# Autodesk Inventor assembly: lançador
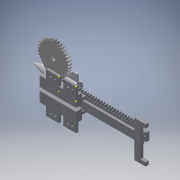
[picture p0: Inventor's stored thumbnail of the model, 180x180]
Saved by Autodesk Inventor 2019 (Build 230136000, 136)
## iProperties
Created: 2018-06-06
Part Number: lançador
Material: Genérico
Document SubType Name: Assembly
Designer: Ernandes
Author: Ernandes
## Documents named in this file (5)
- C:\Users\Ernandes\Google Drive (sguimaraaes@gmail.com)\TCC\3D\lançador.inventor\lançador.inventor\lançador.iam
- C:\Users\Ernandes\Google Drive (sguimaraaes@gmail.com)\TCC\3D\lançador.inventor\lançador.inventor\cremalheira pronta.iam
- C:\Users\Ernandes\Google Drive (sguimaraaes@gmail.com)\TCC\3D\lançador.inventor\foguete.inventor\foguete.iam
- C:\Users\Ernandes\Google Drive (sguimaraaes@gmail.com)\TCC\3D\lançador.inventor\lançador.inventor\suporte p trilho.ipt
- C:\Users\Ernandes\Google Drive (sguimaraaes@gmail.com)\TCC\3D\lançador.inventor\lançador.inventor\suporte p trilho2.ipt
## Components (6 placed, 4 different names)
1. cremalheira pronta:1 [sub-assembly] — Coincidência:8
2. suporte p trilho:1 — Coincidência:3, Coincidência:4
3. suporte p trilho2:1 — Coincidência:1, Coincidência:2
4. suporte p trilho:2 — Coincidência:3, Coincidência:4
5. suporte p trilho2:2 — Coincidência:1, Coincidência:2
6. foguete:2 [sub-assembly] — Coincidência:8
## Relationships (5: Mate 5)
- Coincidência:1 [Mate]: suporte p trilho2:1 ↔ suporte p trilho2:2
- Coincidência:2 [Mate] (40 mm): suporte p trilho2:1 ↔ suporte p trilho2:2
- Coincidência:3 [Mate]: suporte p trilho:1 ↔ suporte p trilho:2
- Coincidência:4 [Mate] (40 mm): suporte p trilho:1 ↔ suporte p trilho:2
- Coincidência:8 [Mate]: cremalheira pronta:1 ↔ foguete:2
